# Autodesk Inventor assembly: RobotArm
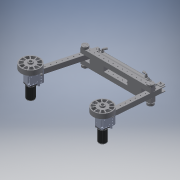
[picture p0: Inventor's stored thumbnail of the model, 180x180]
Saved by Autodesk Inventor 2018 (Build 220112000, 112)
## iProperties
Created: 2018-01-20
Part Number: RobotArm
Document SubType Name: Assembly
Designer: lopez.xavier
Author: lopez.xavier
## Documents named in this file (20)
- \\fs1\studentusers\class19\Lopez.Xavier\documents\RobotArm.iam
- \\fs1\studentusers\class19\Lopez.Xavier\documents\RobotArm Board.ipt
- \\fs1\studentusers\class19\Lopez.Xavier\documents\RobotArm Arm.ipt
- \\fs1\studentusers\class19\Lopez.Xavier\documents\RobotArm Arm2.ipt
- \\fs1\studentusers\class19\Lopez.Xavier\documents\RobotArm Cylinder.ipt
- \\fs1\studentusers\class19\Lopez.Xavier\documents\RobotArm CylinderExtension.ipt
- \\fs1\studentusers\class19\Lopez.Xavier\documents\RobotArm CylinderPart.ipt
- \\fs1\studentusers\class19\Lopez.Xavier\documents\RobotArm Pivot.ipt
- \\fs1\studentusers\class19\Lopez.Xavier\documents\RobotArm ShaftColar.ipt
- \\fs1\studentusers\class19\Lopez.Xavier\documents\RobotArm CylinderPart2.ipt
- \\fs1\studentusers\class19\Lopez.Xavier\documents\RobotArm Nut.ipt
- \\fs1\studentusers\class19\Lopez.Xavier\documents\RobotArm Rivit.ipt
- \\fs1\studentusers\class19\Lopez.Xavier\documents\RobotArm Nut2.ipt
- \\fs1\studentusers\class19\Lopez.Xavier\documents\RobotArm ParallelMount.ipt
- \\fs1\studentusers\class19\Lopez.Xavier\documents\RobotArm Rivet2.ipt
- \\fs1\studentusers\class19\Lopez.Xavier\documents\RobotArm Nut3.ipt
- \\fs1\studentusers\class19\Lopez.Xavier\documents\RobotArm VersaPlanetaryGearbox.iam
- \\fs1\studentusers\class19\Lopez.Xavier\documents\RobotArm Washer.ipt
- \\fs1\studentusers\class19\Lopez.Xavier\documents\RobotArm Wheel.ipt
- \\fs1\studentusers\class19\Lopez.Xavier\documents\RobotArm Washer2.ipt
## Components (38 placed, 19 different names)
1. RobotArm Board:1 — Mate:1, Mate:2, Mate:3, Mate:4, Mate:13, Mate:14, Mate:17, Mate:20, Angle:1, Angle:2
2. RobotArm Arm:1 — Mate:3, Mate:4, Mate:11, Mate:12, Mate:29, Mate:30, Mate:34, Angle:1, Flush:6, Mate:51, Flush:7, Mate:53, Mate:57
3. RobotArm Arm2:1 — Mate:1, Mate:2, Mate:26, Angle:2, Flush:8, Mate:62, Mate:63, Flush:9, Mate:64
4. RobotArm Cylinder:1 — Mate:5, Mate:6, Mate:7, Mate:8, Mate:9, Mate:10, Mate:11, Mate:12
5. RobotArm CylinderExtension:1 — Mate:9, Mate:10, Mate:21, Mate:22, Mate:23, Flush:5
6. RobotArm CylinderPart:1 — Mate:6, Mate:7
7. RobotArm CylinderPart:2 — Mate:5, Mate:8
8. RobotArm Pivot:1 — Mate:13, Flush:1, Mate:15, Mate:16, Flush:2
9. RobotArm Pivot:2 — Mate:14, Flush:3, Flush:4, Mate:18, Mate:19
10. RobotArm ShaftColar:1 — Mate:16, Flush:2
11. RobotArm ShaftColar:2 — Flush:1, Mate:15, Mate:17
12. RobotArm ShaftColar:3 — Flush:3, Mate:18, Mate:20
13. RobotArm ShaftColar:4 — Flush:4, Mate:19
14. RobotArm CylinderPart2:1 — Mate:21, Mate:24, Mate:25, Mate:26, Mate:27, Mate:28, Mate:31
15. RobotArm Nut:1 — Mate:22, Mate:24
16. RobotArm Nut:2 — Mate:23, Mate:25, Flush:5
17. RobotArm Rivit:1 — Mate:29, Mate:30, Mate:33
18. RobotArm Rivit:2 — Mate:27, Mate:28, Mate:32
19. RobotArm Nut2:1 — Mate:31, Mate:32
20. RobotArm Nut2:2 — Mate:33, Mate:34
21. RobotArm ParallelMount:1 — Flush:6, Mate:51, Flush:7, Mate:54, Mate:55, Mate:56, Mate:58, Mate:69, Mate:70, Mate:71, Mate:79
22. RobotArm ParallelMount:2 — Flush:8, Flush:9, Mate:64, Mate:65, Mate:66, Mate:67, Mate:68, Mate:72, Mate:74, Mate:76, Mate:77
23. RobotArm Rivet2:1 — Mate:43, Mate:56, Mate:57
24. RobotArm Rivet2:2 — Mate:44, Mate:53, Mate:55
25. RobotArm Nut3:1 — Mate:43, Mate:58
26. RobotArm Nut3:2 — Mate:44, Mate:54
27. RobotArm Rivet2:3 — Mate:49, Mate:63, Mate:65
28. RobotArm Rivet2:4 — Mate:50, Mate:62, Mate:66
29. RobotArm Nut3:3 — Mate:49, Mate:68
30. RobotArm Nut3:4 — Mate:50, Mate:67
31. RobotArm VersaPlanetaryGearbox:1 [sub-assembly] — Mate:69, Mate:70, Mate:71, Mate:78, Mate:83, Mate:85, Mate:86, Flush:10, Mate:87
32. RobotArm VersaPlanetaryGearbox:2 [sub-assembly] — Mate:72, Mate:74, Mate:75, Mate:76, Mate:80, Mate:82, Flush:11, Mate:88, Mate:89
33. RobotArm Washer:1 — Mate:75, Mate:77, Mate:81
34. RobotArm Washer:2 — Mate:78, Mate:79, Mate:84
35. RobotArm Wheel:1 — Mate:83, Mate:84, Mate:85
36. RobotArm Wheel:2 — Mate:80, Mate:81, Mate:82
37. RobotArm Washer2:1 — Mate:86, Flush:10, Mate:87
38. RobotArm Washer2:2 — Flush:11, Mate:88, Mate:89
## Relationships (85: Mate 72, Flush 11, Angle 2)
- Mate:1: RobotArm Board:1 ↔ RobotArm Arm2:1
- Mate:2: RobotArm Board:1 ↔ RobotArm Arm2:1
- Mate:3: RobotArm Board:1 ↔ RobotArm Arm:1
- Mate:4: RobotArm Board:1 ↔ RobotArm Arm:1
- Mate:5: RobotArm Cylinder:1 ↔ RobotArm CylinderPart:2
- Mate:6: RobotArm Cylinder:1 ↔ RobotArm CylinderPart:1
- Mate:7: RobotArm Cylinder:1 ↔ RobotArm CylinderPart:1
- Mate:8: RobotArm Cylinder:1 ↔ RobotArm CylinderPart:2
- Mate:9: RobotArm Cylinder:1 ↔ RobotArm CylinderExtension:1
- Mate:10: RobotArm Cylinder:1 ↔ RobotArm CylinderExtension:1
- Mate:11: RobotArm Arm:1 ↔ RobotArm Cylinder:1
- Mate:12 (5.08 mm): RobotArm Arm:1 ↔ RobotArm Cylinder:1
- Mate:13: RobotArm Board:1 ↔ RobotArm Pivot:1
- Mate:14: RobotArm Board:1 ↔ RobotArm Pivot:2
- Flush:1: RobotArm Pivot:1 ↔ RobotArm ShaftColar:2
- Mate:15: RobotArm Pivot:1 ↔ RobotArm ShaftColar:2
- Mate:16: RobotArm Pivot:1 ↔ RobotArm ShaftColar:1
- Flush:2: RobotArm Pivot:1 ↔ RobotArm ShaftColar:1
- Mate:17: RobotArm Board:1 ↔ RobotArm ShaftColar:2
- Flush:3: RobotArm Pivot:2 ↔ RobotArm ShaftColar:3
- Flush:4: RobotArm Pivot:2 ↔ RobotArm ShaftColar:4
- Mate:18: RobotArm Pivot:2 ↔ RobotArm ShaftColar:3
- Mate:19: RobotArm Pivot:2 ↔ RobotArm ShaftColar:4
- Mate:20: RobotArm Board:1 ↔ RobotArm ShaftColar:3
- Mate:21: RobotArm CylinderExtension:1 ↔ RobotArm CylinderPart2:1
- Mate:22: RobotArm CylinderExtension:1 ↔ RobotArm Nut:1
- Mate:23: RobotArm CylinderExtension:1 ↔ RobotArm Nut:2
- Mate:24: RobotArm CylinderPart2:1 ↔ RobotArm Nut:1
- Mate:25: RobotArm CylinderPart2:1 ↔ RobotArm Nut:2
- Flush:5: RobotArm CylinderExtension:1 ↔ RobotArm Nut:2
- Mate:26: RobotArm Arm2:1 ↔ RobotArm CylinderPart2:1
- Mate:27: RobotArm CylinderPart2:1 ↔ RobotArm Rivit:2
- Mate:28: RobotArm CylinderPart2:1 ↔ RobotArm Rivit:2
- Mate:29: RobotArm Arm:1 ↔ RobotArm Rivit:1
- Mate:30: RobotArm Arm:1 ↔ RobotArm Rivit:1
- Mate:31: RobotArm CylinderPart2:1 ↔ RobotArm Nut2:1
- Mate:32: RobotArm Rivit:2 ↔ RobotArm Nut2:1
- Mate:33: RobotArm Rivit:1 ↔ RobotArm Nut2:2
- Mate:34: RobotArm Arm:1 ↔ RobotArm Nut2:2
- Angle:1 (90 deg): RobotArm Board:1 ↔ RobotArm Arm:1
- Angle:2 (90 deg): RobotArm Board:1 ↔ RobotArm Arm2:1
- Mate:43: RobotArm Rivet2:1 ↔ RobotArm Nut3:1
- Mate:44: RobotArm Rivet2:2 ↔ RobotArm Nut3:2
- Mate:49: RobotArm Rivet2:3 ↔ RobotArm Nut3:3
- Mate:50: RobotArm Rivet2:4 ↔ RobotArm Nut3:4
- Flush:6: RobotArm Arm:1 ↔ RobotArm ParallelMount:1
- Mate:51: RobotArm Arm:1 ↔ RobotArm ParallelMount:1
- Flush:7: RobotArm Arm:1 ↔ RobotArm ParallelMount:1
- Flush:8: RobotArm Arm2:1 ↔ RobotArm ParallelMount:2
- Mate:53: RobotArm Arm:1 ↔ RobotArm Rivet2:2
- Mate:54: RobotArm ParallelMount:1 ↔ RobotArm Nut3:2
- Mate:55: RobotArm ParallelMount:1 ↔ RobotArm Rivet2:2
- Mate:56: RobotArm ParallelMount:1 ↔ RobotArm Rivet2:1
- Mate:57: RobotArm Arm:1 ↔ RobotArm Rivet2:1
- Mate:58: RobotArm ParallelMount:1 ↔ RobotArm Nut3:1
- Mate:62: RobotArm Arm2:1 ↔ RobotArm Rivet2:4
- Mate:63: RobotArm Arm2:1 ↔ RobotArm Rivet2:3
- Flush:9: RobotArm Arm2:1 ↔ RobotArm ParallelMount:2
- Mate:64: RobotArm Arm2:1 ↔ RobotArm ParallelMount:2
- Mate:65: RobotArm ParallelMount:2 ↔ RobotArm Rivet2:3
- Mate:66: RobotArm ParallelMount:2 ↔ RobotArm Rivet2:4
- Mate:67: RobotArm ParallelMount:2 ↔ RobotArm Nut3:4
- Mate:68: RobotArm ParallelMount:2 ↔ RobotArm Nut3:3
- Mate:69: RobotArm ParallelMount:1 ↔ RobotArm VersaPlanetaryGearbox:1
- Mate:70: RobotArm ParallelMount:1 ↔ RobotArm VersaPlanetaryGearbox:1
- Mate:71: RobotArm ParallelMount:1 ↔ RobotArm VersaPlanetaryGearbox:1
- Mate:72: RobotArm ParallelMount:2 ↔ RobotArm VersaPlanetaryGearbox:2
- Mate:74: RobotArm ParallelMount:2 ↔ RobotArm VersaPlanetaryGearbox:2
- Mate:75: RobotArm VersaPlanetaryGearbox:2 ↔ RobotArm Washer:1
- Mate:76: RobotArm ParallelMount:2 ↔ RobotArm VersaPlanetaryGearbox:2
- Mate:77: RobotArm ParallelMount:2 ↔ RobotArm Washer:1
- Mate:78: RobotArm VersaPlanetaryGearbox:1 ↔ RobotArm Washer:2
- Mate:79: RobotArm ParallelMount:1 ↔ RobotArm Washer:2
- Mate:80: RobotArm VersaPlanetaryGearbox:2 ↔ RobotArm Wheel:2
- Mate:81: RobotArm Washer:1 ↔ RobotArm Wheel:2
- Mate:82: RobotArm VersaPlanetaryGearbox:2 ↔ RobotArm Wheel:2
- Mate:83: RobotArm VersaPlanetaryGearbox:1 ↔ RobotArm Wheel:1
- Mate:84: RobotArm Washer:2 ↔ RobotArm Wheel:1
- Mate:85: RobotArm VersaPlanetaryGearbox:1 ↔ RobotArm Wheel:1
- Mate:86: RobotArm VersaPlanetaryGearbox:1 ↔ RobotArm Washer2:1
- Flush:10: RobotArm VersaPlanetaryGearbox:1 ↔ RobotArm Washer2:1
- Mate:87: RobotArm VersaPlanetaryGearbox:1 ↔ RobotArm Washer2:1
- Flush:11: RobotArm VersaPlanetaryGearbox:2 ↔ RobotArm Washer2:2
- Mate:88: RobotArm VersaPlanetaryGearbox:2 ↔ RobotArm Washer2:2
- Mate:89: RobotArm VersaPlanetaryGearbox:2 ↔ RobotArm Washer2:2
